# Autodesk Inventor assembly: Sessao5_0002
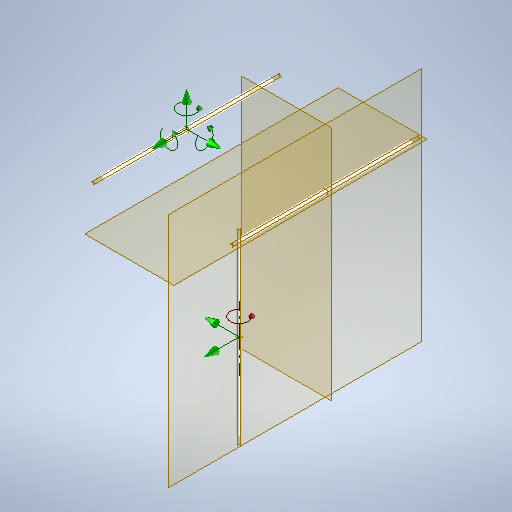
[picture p0: Inventor's stored thumbnail of the model, 512x512]
Saved by Autodesk Inventor 2025.2 (Build 292293000, 293)
## iProperties
Created: 2025-03-28
Part Number: Sessao5_0002
Document SubType Name: Assembly
Designer: lucas
Author: lucas
## Documents named in this file (2)
- C:\Users\lucas\OneDrive\Documentos\Documentos\Gustavo\Mozangao\Robotica_Fundamentos\Inventor\Sessao5\Sessao5_0002.iam
- C:\Users\lucas\OneDrive\Documentos\Documentos\Gustavo\Mozangao\Robotica_Fundamentos\Inventor\Sessao5\20×20 4 slots profile_AST02002004.ipt
## Components (3 placed, 1 different names)
1. 20×20 4 slots profile_AST02002004:1 — Alinhado:1, Alinhado:2, Alinhado:3, Alinhado:4
2. 20×20 4 slots profile_AST02002004:2 — Alinhado:4
3. 20×20 4 slots profile_AST02002004:3
## Relationships (4: Flush 4)
- Alinhado:1 [Flush]: 20×20 4 slots profile_AST02002004:1
- Alinhado:2 [Flush]: 20×20 4 slots profile_AST02002004:1
- Alinhado:3 [Flush]: 20×20 4 slots profile_AST02002004:1
- Alinhado:4 [Flush]: 20×20 4 slots profile_AST02002004:1 ↔ 20×20 4 slots profile_AST02002004:2
